# Autodesk Inventor assembly: МД.001.100 - База поворотного стола
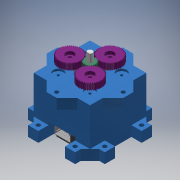
[picture p0: Inventor's stored thumbnail of the model, 180x180]
Saved by Autodesk Inventor 2019 (Build 230136000, 136)
## iProperties
Created: 2019-12-22
Part Number: МД.001.100 - База поворотного стола
Material: Типовые
Document SubType Name: Assembly
Designer: Петров Иван
Author: Петров Иван
## Documents named in this file (6)
- E:\IVAN\Ivan_desktop\GitHub\Arm_manip\hardware\МД.001.100 - База поворотного стола.iam
- E:\IVAN\Ivan_desktop\GitHub\Arm_manip\hardware\МД.001.101 - Стойка мотора.ipt
- E:\IVAN\Ivan_desktop\GitHub\Arm_manip\hardware\Standart_things\Nema 17HS4401-S.ipt
- E:\IVAN\Ivan_desktop\GitHub\Arm_manip\hardware\МД.001.203 - Водило.ipt
- E:\IVAN\Ivan_desktop\GitHub\Arm_manip\hardware\МД.001.204 - Солнечная шестерня.ipt
- E:\IVAN\Ivan_desktop\GitHub\Arm_manip\hardware\МД.001.203 - Сателлит.ipt
## Components (7 placed, 5 different names)
1. МД.001.101 - Стойка мотора:1 — Совмещение:1, Совмещение:2, Совмещение:3, Совмещение:15
2. Nema 17HS4401-S:1 — Совмещение:1, Совмещение:2, Совмещение:3, Совмещение:14, Совмещение:23
3. МД.001.203 - Водило:1 — Совмещение:14, Совмещение:15, Совмещение:22, Совмещение:24, Совмещение:25, Совмещение:26, Совмещение:27, Совмещение:28, Совмещение:29
4. МД.001.204 - Солнечная шестерня:1 — Совмещение:22, Совмещение:23
5. Цилиндрическое зубчатое зацепление1:1 — Совмещение:24, Совмещение:25
6. Цилиндрическое зубчатое зацепление1:2 — Совмещение:26, Совмещение:27
7. Цилиндрическое зубчатое зацепление1:3 — Совмещение:28, Совмещение:29
## Relationships (13: Mate 13)
- Совмещение:1 [Mate]: МД.001.101 - Стойка мотора:1 ↔ Nema 17HS4401-S:1
- Совмещение:2 [Mate]: МД.001.101 - Стойка мотора:1 ↔ Nema 17HS4401-S:1
- Совмещение:3 [Mate]: МД.001.101 - Стойка мотора:1 ↔ Nema 17HS4401-S:1
- Совмещение:14 [Mate]: Nema 17HS4401-S:1 ↔ МД.001.203 - Водило:1
- Совмещение:15 [Mate]: МД.001.101 - Стойка мотора:1 ↔ МД.001.203 - Водило:1
- Совмещение:22 [Mate]: МД.001.203 - Водило:1 ↔ МД.001.204 - Солнечная шестерня:1
- Совмещение:23 [Mate]: Nema 17HS4401-S:1 ↔ МД.001.204 - Солнечная шестерня:1
- Совмещение:24 [Mate]: МД.001.203 - Водило:1 ↔ Цилиндрическое зубчатое зацепление1:1
- Совмещение:25 [Mate]: МД.001.203 - Водило:1 ↔ Цилиндрическое зубчатое зацепление1:1
- Совмещение:26 [Mate]: МД.001.203 - Водило:1 ↔ Цилиндрическое зубчатое зацепление1:2
- Совмещение:27 [Mate]: МД.001.203 - Водило:1 ↔ Цилиндрическое зубчатое зацепление1:2
- Совмещение:28 [Mate]: МД.001.203 - Водило:1 ↔ Цилиндрическое зубчатое зацепление1:3
- Совмещение:29 [Mate]: МД.001.203 - Водило:1 ↔ Цилиндрическое зубчатое зацепление1:3
